# Autodesk Inventor assembly: Assembly2
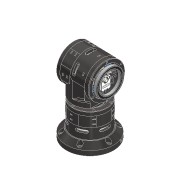
[picture p0: Inventor's stored thumbnail of the model, 180x180]
Saved by Autodesk Inventor 2021 (Build 250183000, 183)
## iProperties
Created: 2020-08-06
Part Number: Assembly2
Document SubType Name: Assembly
Designer: Derm
Author: Derm
## Documents named in this file (3)
- C:\Users\Derm\roboticArm\hardware\v9\Assembly2.iam
- C:\Users\Derm\roboticArm\hardware\v9\j0.iam
- C:\Users\Derm\roboticArm\hardware\v9\j1.iam
## Components (2 placed, 2 different names)
1. j0:1 [sub-assembly] — Mate:1, Mate:2
2. j1:1 [sub-assembly] — Mate:2
## Relationships (2: Mate 2)
- Mate:1: j0:1
- Mate:2: j0:1 ↔ j1:1
